# Autodesk Inventor assembly: assembled cover
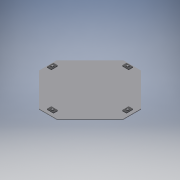
[picture p0: Inventor's stored thumbnail of the model, 180x180]
Saved by Autodesk Inventor 2016 (Build 200138000, 138)
## iProperties
Created: 2016-07-21
Part Number: assembled cover
Document SubType Name: Assembly
Designer: Jonathan
Author: Jonathan
## Documents named in this file (3)
- C:\Users\Jonathan\Desktop\Models\Four Paddle Detector\frame\separator\assembled cover.iam
- C:\Users\Jonathan\Desktop\Models\Four Paddle Detector\frame\separator\separatingPanels.ipt
- C:\Users\Jonathan\Desktop\Models\Four Paddle Detector\frame\brackets\m5x6 assembly.iam
## Components (5 placed, 2 different names)
1. separatingPanels:1 — Angle:1, Angle:2, Angle:3, Angle:4, Mate:2, Mate:3, Mate:4, Mate:5, Mate:6, Mate:7, Mate:8
2. m5x6 assembly:1 [sub-assembly] — Angle:1, Mate:4, Flush:1
3. m5x6 assembly:2 [sub-assembly] — Angle:2, Mate:3, Mate:8
4. m5x6 assembly:3 [sub-assembly] — Angle:4, Mate:5, Flush:1, Mate:6
5. m5x6 assembly:4 [sub-assembly] — Angle:3, Mate:2, Mate:7
## Relationships (12: Mate 7, Angle 4, Flush 1)
- Angle:1 (0 deg): separatingPanels:1 ↔ m5x6 assembly:1
- Angle:2 (0 deg): separatingPanels:1 ↔ m5x6 assembly:2
- Angle:3 (0 deg): separatingPanels:1 ↔ m5x6 assembly:4
- Angle:4 (0 deg): separatingPanels:1 ↔ m5x6 assembly:3
- Mate:2: separatingPanels:1 ↔ m5x6 assembly:4
- Mate:3: separatingPanels:1 ↔ m5x6 assembly:2
- Mate:4: separatingPanels:1 ↔ m5x6 assembly:1
- Mate:5: separatingPanels:1 ↔ m5x6 assembly:3
- Flush:1: m5x6 assembly:1 ↔ m5x6 assembly:3
- Mate:6: separatingPanels:1 ↔ m5x6 assembly:3
- Mate:7: separatingPanels:1 ↔ m5x6 assembly:4
- Mate:8: separatingPanels:1 ↔ m5x6 assembly:2
